# Autodesk Inventor assembly: 弹簧
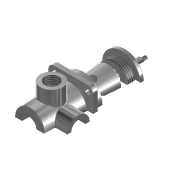
[picture p0: Inventor's stored thumbnail of the model, 180x180]
Saved by Autodesk Inventor 2022 (Build 260153000, 153)
## iProperties
Created: 2023-03-15
Part Number: 弹簧
Document SubType Name: Assembly
Designer: Lzy18
Author: Lzy18
## Documents named in this file (5)
- C:\Users\Lzy18\Desktop\20工2\弹簧.iam
- C:\Users\Lzy18\Desktop\20工2\阀体.ipt
- C:\Users\Lzy18\Desktop\20工2\旋塞.ipt
- C:\Users\Lzy18\Desktop\20工2\塞杆.ipt
- C:\Users\Lzy18\Desktop\20工2\螺盖.ipt
## Components (4 placed, 4 different names)
1. 阀体:1 — 配合:1
2. 旋塞:1 — 配合:1, 配合:2, 配合:3
3. 塞杆:1 — 配合:2, 配合:3, 配合:4, 配合:5
4. 螺盖:1 — 配合:4, 配合:5
## Relationships (5: Mate 5)
- 配合:1 [Mate]: 阀体:1 ↔ 旋塞:1
- 配合:2 [Mate]: 旋塞:1 ↔ 塞杆:1
- 配合:3 [Mate]: 旋塞:1 ↔ 塞杆:1
- 配合:4 [Mate]: 塞杆:1 ↔ 螺盖:1
- 配合:5 [Mate] (33.5 mm): 塞杆:1 ↔ 螺盖:1
